# Autodesk Inventor assembly: ASY ДМФ 0100 Барабан v2.0
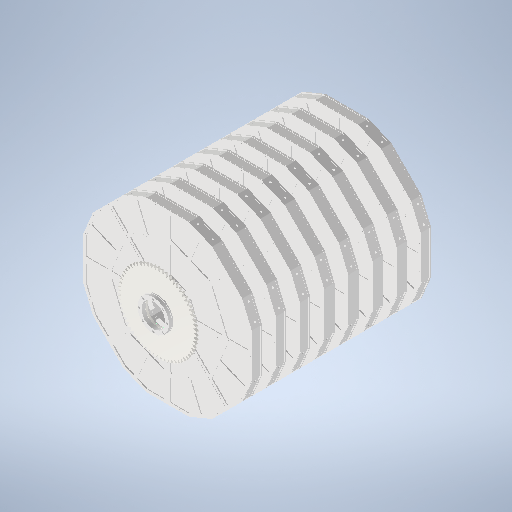
[picture p0: Inventor's stored thumbnail of the model, 512x512]
Saved by Autodesk Inventor 2025 (Build 290162010, 162A)
## iProperties
Created: 2024-04-28
Part Number: ASY ДМФ 0100 Барабан v2.0
Document SubType Name: Assembly
Designer: pokla
Author: pokla
## Documents named in this file (14)
- C:\Users\pokla\Documents\Inventor\ДФО\ДМФ\DMF-Disk-Micro-Filter\ASY ДМФ 0100 Барабан v2.0.iam
- C:\Users\pokla\Documents\Inventor\ДФО\ДМФ\DMF-Disk-Micro-Filter\ДМФ 01 21 Барабан торец НОС v2.0.ipt
- C:\Users\pokla\Documents\Inventor\ДФО\ДМФ\DMF-Disk-Micro-Filter\ДМФ 01 13 Барабан Лист лев брт v2.0.ipt
- C:\Users\pokla\Documents\Inventor\ДФО\ДМФ\DMF-Disk-Micro-Filter\ДМФ 01 14 Барабан Лист прав брт v2.0.ipt
- C:\Users\pokla\Documents\Inventor\ДФО\ДМФ\DMF-Disk-Micro-Filter\ДМФ 01 31 Барабан Опорное кольцо НОС v2.0.ipt
- C:\Users\pokla\Documents\Inventor\ДФО\ДМФ\DMF-Disk-Micro-Filter\ДМФ 01 17 опора крышки v2.0.ipt
- C:\Users\pokla\Documents\Inventor\ДФО\ДМФ\DMF-Disk-Micro-Filter\ДМФ 000 размеры v2.0.ipt
- C:\Users\pokla\Documents\Inventor\ДФО\ДМФ\DMF-Disk-Micro-Filter\ДМФ 01 41 Шестерня ведомая v2.0.ipt
- C:\Users\pokla\Documents\Inventor\ДФО\ДМФ\DMF-Disk-Micro-Filter\ДМФ 01 12 Барабан усилитель v2.0.ipt
- C:\Users\pokla\Documents\Inventor\ДФО\ДМФ\DMF-Disk-Micro-Filter\ASY ДМФ 010 крышка v2.0.iam
- C:\Users\pokla\Documents\Inventor\ДФО\ДМФ\DMF-Disk-Micro-Filter\ДМФ 01 32 Барабан Опорное кольцо КОРМА v2.0.ipt
- C:\Users\pokla\Documents\Inventor\ДФО\ДМФ\DMF-Disk-Micro-Filter\ДМФ 01 22 Барабан торец КОРМА v2.0.ipt
- C:\Users\pokla\Documents\Inventor\ДФО\ДМФ\DMF-Disk-Micro-Filter\ASY фильтр пакет v2.0.iam
- C:\Users\pokla\Documents\Inventor\ДФО\ДМФ\DMF-Disk-Micro-Filter\DMF v2.0\ДМФ 01 21 Барабан торец НОС.ipt
## Components (68 placed, 13 different names)
1. ДМФ 000 размеры v2.0:1
2. ДМФ 01 21 Барабан торец НОС v2.0:2 — Mate:15, Flush:8, Flush:9, Flush:10, Flush:11, Mate:16, Mate:17, Rigid:19, Mate:19, Mate:21, Flush:15, Flush:16, Flush:17, Mate:23
3. ДМФ 01 31 Барабан Опорное кольцо НОС v2.0:1 — Rotational:1
4. ДМФ 01 32 Барабан Опорное кольцо КОРМА v2.0:1 — Rigid:20
5. ДМФ 01 22 Барабан торец КОРМА v2.0:1 — Flush:12, Flush:13, Mate:18, Rigid:20
6. ДМФ 01 13 Барабан Лист лев брт v2.0:1 — Mate:12, Flush:7, Flush:10, Flush:11, Mate:16, Flush:13, Mate:18, Mate:20, Mate:29
7. ДМФ 01 14 Барабан Лист прав брт v2.0:1 — Mate:11, Flush:8, Flush:9, Mate:17, Flush:12, Mate:22, Mate:28
8. ДМФ 01 17 опора крышки v2.0:1 — Mate:21, Flush:15, Mate:22
9. ДМФ 01 17 опора крышки v2.0:2 — Mate:19, Mate:20, Mate:27
10. ДМС 105 Шестерня ведомая:1 — Rigid:19, Rotational:1
11. ASY ДМФ 010 крышка v2.0:1 [sub-assembly] — Flush:16, Flush:17, Mate:23, Mate:27
12. ДМФ 01 29 Барабан сборочный лист:1 — Mate:28, Mate:29
13. ДМФ 01 12 Барабан усилитель v2.0:4 — Rigid:10
14. ДМФ 01 12 Барабан усилитель v2.0:1 — Rigid:8
15. ДМФ 01 12 Барабан усилитель v2.0:5 — Rigid:10, Rigid:11, Rigid:14
16. ДМФ 01 12 Барабан усилитель v2.0:2 — Rigid:8, Rigid:9, Rigid:14
17. ДМФ 01 12 Барабан усилитель v2.0:3 — Rigid:9, Mate:12
18. ДМФ 01 12 Барабан усилитель v2.0:6 — Rigid:11
19. ДМФ 01 12 Барабан усилитель v2.0:7
20. ДМФ 01 12 Барабан усилитель v2.0:8
21. ДМФ 01 12 Барабан усилитель v2.0:21
22. ДМФ 01 12 Барабан усилитель v2.0:28
23. ДМФ 01 12 Барабан усилитель v2.0:35
24. ДМФ 01 12 Барабан усилитель v2.0:42
25. ДМФ 01 12 Барабан усилитель v2.0:9
26. ДМФ 01 12 Барабан усилитель v2.0:10
27. ДМФ 01 12 Барабан усилитель v2.0:22
28. ДМФ 01 12 Барабан усилитель v2.0:29
29. ДМФ 01 12 Барабан усилитель v2.0:36
30. ДМФ 01 12 Барабан усилитель v2.0:43
31. ДМФ 01 12 Барабан усилитель v2.0:11
32. ДМФ 01 12 Барабан усилитель v2.0:12
33. ДМФ 01 12 Барабан усилитель v2.0:23
34. ДМФ 01 12 Барабан усилитель v2.0:30
35. ДМФ 01 12 Барабан усилитель v2.0:37
36. ДМФ 01 12 Барабан усилитель v2.0:44
37. ДМФ 01 12 Барабан усилитель v2.0:13
38. ДМФ 01 12 Барабан усилитель v2.0:14
39. ДМФ 01 12 Барабан усилитель v2.0:24
40. ДМФ 01 12 Барабан усилитель v2.0:31
41. ДМФ 01 12 Барабан усилитель v2.0:38
42. ДМФ 01 12 Барабан усилитель v2.0:45
43. ДМФ 01 12 Барабан усилитель v2.0:15
44. ДМФ 01 12 Барабан усилитель v2.0:16
45. ДМФ 01 12 Барабан усилитель v2.0:25
46. ДМФ 01 12 Барабан усилитель v2.0:32
47. ДМФ 01 12 Барабан усилитель v2.0:39
48. ДМФ 01 12 Барабан усилитель v2.0:46
49. ДМФ 01 12 Барабан усилитель v2.0:17
50. ДМФ 01 12 Барабан усилитель v2.0:18
51. ДМФ 01 12 Барабан усилитель v2.0:26
52. ДМФ 01 12 Барабан усилитель v2.0:33
53. ДМФ 01 12 Барабан усилитель v2.0:40
54. ДМФ 01 12 Барабан усилитель v2.0:47
55. ДМФ 01 12 Барабан усилитель v2.0:19 — Mate:11
56. ДМФ 01 12 Барабан усилитель v2.0:20
57. ДМФ 01 12 Барабан усилитель v2.0:27
58. ДМФ 01 12 Барабан усилитель v2.0:34
59. ДМФ 01 12 Барабан усилитель v2.0:41
60. ДМФ 01 12 Барабан усилитель v2.0:48 — Flush:7, Mate:26
61. ASY фильтр пакет v2.0:1 [sub-assembly] — Mate:24, Mate:25, Mate:26
62. ASY фильтр пакет v2.0:2 [sub-assembly]
63. ASY фильтр пакет v2.0:3 [sub-assembly]
64. ASY фильтр пакет v2.0:4 [sub-assembly]
65. ASY фильтр пакет v2.0:5 [sub-assembly]
66. ASY фильтр пакет v2.0:6 [sub-assembly]
67. ASY фильтр пакет v2.0:7 [sub-assembly]
68. ASY фильтр пакет v2.0:8 [sub-assembly]
## Component patterns: (8 elements, first: ДМФ 01 12 Барабан усилитель v2.0:4 + ДМФ 01 12 Барабан усилитель v2.0:1 + ДМФ 01 12 Барабан усилитель v2.0:5 + ДМФ 01 12 Барабан усилитель v2.0:2 + ДМФ 01 12 Барабан усилитель v2.0:3 + ДМФ 01 12 Барабан усилитель v2.0:6), (8 elements, first: ASY фильтр пакет v2.0:1)
## Relationships (35: Mate 17, Flush 10, WeldJoint 7, RevoluteJoint 1)
- Rigid:8 [WeldJoint]: ДМФ 01 12 Барабан усилитель v2.0:1 ↔ ДМФ 01 12 Барабан усилитель v2.0:2
- Rigid:9 [WeldJoint]: ДМФ 01 12 Барабан усилитель v2.0:2 ↔ ДМФ 01 12 Барабан усилитель v2.0:3
- Rigid:10 [WeldJoint]: ДМФ 01 12 Барабан усилитель v2.0:4 ↔ ДМФ 01 12 Барабан усилитель v2.0:5
- Rigid:11 [WeldJoint]: ДМФ 01 12 Барабан усилитель v2.0:5 ↔ ДМФ 01 12 Барабан усилитель v2.0:6
- Rigid:14 [WeldJoint] (108 mm): ДМФ 01 12 Барабан усилитель v2.0:5 ↔ ДМФ 01 12 Барабан усилитель v2.0:2
- Mate:11: ДМФ 01 14 Барабан Лист прав брт v2.0:1 ↔ ДМФ 01 12 Барабан усилитель v2.0:19
- Mate:12: ДМФ 01 13 Барабан Лист лев брт v2.0:1 ↔ ДМФ 01 12 Барабан усилитель v2.0:3
- Flush:7 (29 mm): ДМФ 01 13 Барабан Лист лев брт v2.0:1 ↔ ДМФ 01 12 Барабан усилитель v2.0:48
- Mate:15: ДМФ 01 21 Барабан торец НОС v2.0:2
- Flush:8: ДМФ 01 21 Барабан торец НОС v2.0:2 ↔ ДМФ 01 14 Барабан Лист прав брт v2.0:1
- Flush:9: ДМФ 01 21 Барабан торец НОС v2.0:2 ↔ ДМФ 01 14 Барабан Лист прав брт v2.0:1
- Flush:10: ДМФ 01 21 Барабан торец НОС v2.0:2 ↔ ДМФ 01 13 Барабан Лист лев брт v2.0:1
- Flush:11: ДМФ 01 21 Барабан торец НОС v2.0:2 ↔ ДМФ 01 13 Барабан Лист лев брт v2.0:1
- Mate:16: ДМФ 01 21 Барабан торец НОС v2.0:2 ↔ ДМФ 01 13 Барабан Лист лев брт v2.0:1
- Mate:17: ДМФ 01 21 Барабан торец НОС v2.0:2 ↔ ДМФ 01 14 Барабан Лист прав брт v2.0:1
- Flush:12: ДМФ 01 22 Барабан торец КОРМА v2.0:1 ↔ ДМФ 01 14 Барабан Лист прав брт v2.0:1
- Flush:13: ДМФ 01 22 Барабан торец КОРМА v2.0:1 ↔ ДМФ 01 13 Барабан Лист лев брт v2.0:1
- Mate:18: ДМФ 01 22 Барабан торец КОРМА v2.0:1 ↔ ДМФ 01 13 Барабан Лист лев брт v2.0:1
- Rigid:19 [WeldJoint]: ДМФ 01 21 Барабан торец НОС v2.0:2 ↔ ДМС 105 Шестерня ведомая:1
- Rotational:1 [RevoluteJoint]: ДМФ 01 31 Барабан Опорное кольцо НОС v2.0:1 ↔ ДМС 105 Шестерня ведомая:1
- Mate:19: ДМФ 01 21 Барабан торец НОС v2.0:2 ↔ ДМФ 01 17 опора крышки v2.0:2
- Mate:20: ДМФ 01 13 Барабан Лист лев брт v2.0:1 ↔ ДМФ 01 17 опора крышки v2.0:2
- Mate:21: ДМФ 01 21 Барабан торец НОС v2.0:2 ↔ ДМФ 01 17 опора крышки v2.0:1
- Flush:15 (-2 mm): ДМФ 01 21 Барабан торец НОС v2.0:2 ↔ ДМФ 01 17 опора крышки v2.0:1
- Mate:22: ДМФ 01 14 Барабан Лист прав брт v2.0:1 ↔ ДМФ 01 17 опора крышки v2.0:1
- Flush:16: ДМФ 01 21 Барабан торец НОС v2.0:2 ↔ ASY ДМФ 010 крышка v2.0:1
- Flush:17: ДМФ 01 21 Барабан торец НОС v2.0:2 ↔ ASY ДМФ 010 крышка v2.0:1
- Mate:23: ДМФ 01 21 Барабан торец НОС v2.0:2 ↔ ASY ДМФ 010 крышка v2.0:1
- Mate:24: ASY фильтр пакет v2.0:1
- Mate:25: ASY фильтр пакет v2.0:1
- Mate:26: ДМФ 01 12 Барабан усилитель v2.0:48 ↔ ASY фильтр пакет v2.0:1
- Mate:27: ДМФ 01 17 опора крышки v2.0:2 ↔ ASY ДМФ 010 крышка v2.0:1
- Mate:28: ДМФ 01 14 Барабан Лист прав брт v2.0:1 ↔ ДМФ 01 29 Барабан сборочный лист:1
- Mate:29: ДМФ 01 13 Барабан Лист лев брт v2.0:1 ↔ ДМФ 01 29 Барабан сборочный лист:1
- Rigid:20 [WeldJoint]: ДМФ 01 32 Барабан Опорное кольцо КОРМА v2.0:1 ↔ ДМФ 01 22 Барабан торец КОРМА v2.0:1
